# Autodesk Inventor assembly: LEAP ASS
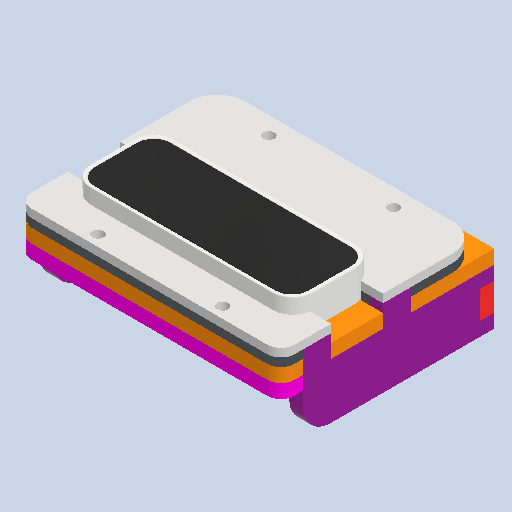
[picture p0: Inventor's stored thumbnail of the model, 512x512]
Saved by Autodesk Inventor 2022 (Build 260153000, 153)
## iProperties
Created: 2021-06-18
Part Number: LEAP ASS
Document SubType Name: Assembly
Designer: benka
Author: benka
## Documents named in this file (8)
- C:\Users\benka\Downloads\Sleeker Design\Leap Holder\LEAP ASS.iam
- C:\Users\benka\Downloads\Sleeker Design\Leap Holder\spacer.ipt
- C:\Users\benka\Downloads\Sleeker Design\Leap Holder\spacer top.ipt
- C:\Users\benka\Downloads\Sleeker Design\Leap Holder\Bottom Base.ipt
- C:\Users\benka\Downloads\Sleeker Design\Leap Holder\AP.ipt
- C:\Users\benka\Downloads\Sleeker Design\Leap Holder\Top Base.ipt
- C:\Users\benka\Downloads\Sleeker Design\Leap Holder\Side.ipt
- C:\Users\benka\Downloads\Sleeker Design\Leap Holder\leap_motion.ipt
## Components (8 placed, 7 different names)
1. spacer:1 — Flush:2, Mate:11, Flush:3, Mate:12, Flush:4, Flush:5
2. spacer top:1 — Mate:12, Flush:4, Flush:5, Mate:17
3. Bottom Base:1 — Flush:1, Mate:1, Mate:8, Mate:9
4. AP:1 — Mate:8, Mate:9, Mate:10, Mate:14, Mate:15, Flush:6, Mate:16, Flush:7, Flush:8
5. Top Base:1 — Flush:1, Mate:1, Mate:10, Flush:2, Mate:11, Flush:3, Mate:13
6. Side:1 — Mate:16, Flush:7, Flush:8
7. Side:2 — Mate:14, Mate:15, Flush:6
8. leap_motion:1 — Mate:13, Mate:17
## Relationships (19: Mate 11, Flush 8)
- Flush:1: Bottom Base:1 ↔ Top Base:1
- Mate:1: Bottom Base:1 ↔ Top Base:1
- Mate:8: Bottom Base:1 ↔ AP:1
- Mate:9: Bottom Base:1 ↔ AP:1
- Mate:10: AP:1 ↔ Top Base:1
- Flush:2: spacer:1 ↔ Top Base:1
- Mate:11: spacer:1 ↔ Top Base:1
- Flush:3: spacer:1 ↔ Top Base:1
- Mate:12: spacer:1 ↔ spacer top:1
- Flush:4: spacer:1 ↔ spacer top:1
- Flush:5: spacer:1 ↔ spacer top:1
- Mate:13: Top Base:1 ↔ leap_motion:1
- Mate:14: AP:1 ↔ Side:2
- Mate:15: AP:1 ↔ Side:2
- Flush:6: AP:1 ↔ Side:2
- Mate:16: AP:1 ↔ Side:1
- Flush:7: AP:1 ↔ Side:1
- Flush:8: AP:1 ↔ Side:1
- Mate:17: spacer top:1 ↔ leap_motion:1
